# Autodesk Inventor assembly: ToolBox with Handle
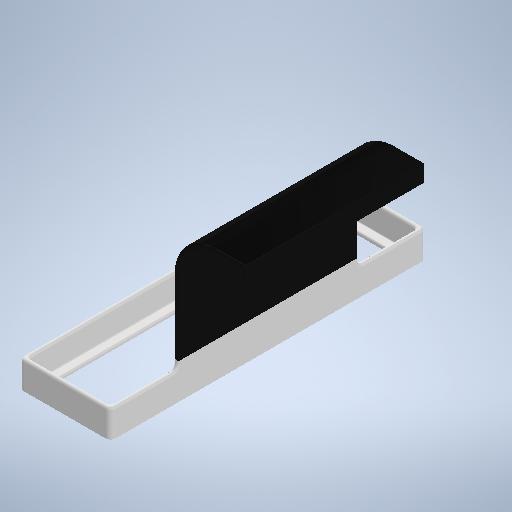
[picture p0: Inventor's stored thumbnail of the model, 512x512]
Saved by Autodesk Inventor 2025 (Build 290162000, 162)
## iProperties
Created: 2024-11-06
Part Number: ToolBox with Handle
Document SubType Name: Assembly
Designer: Makusimu
Author: Makusimu
## Documents named in this file (3)
- Z:\#3D models\Подставка для инструментов\ToolBox with Handle.iam
- Z:\#3D models\Подставка для инструментов\Case for ToolBox.ipt
- Z:\#3D models\Подставка для инструментов\Handle.ipt
## Components (2 placed, 2 different names)
1. Case for ToolBox:1 — Совмещение:1, Заподлицо:1
2. Handle:1 — Совмещение:1, Заподлицо:1
## Relationships (2: Mate 1, Flush 1)
- Совмещение:1 [Mate]: Case for ToolBox:1 ↔ Handle:1
- Заподлицо:1 [Flush]: Case for ToolBox:1 ↔ Handle:1
